# Autodesk Inventor assembly: Support
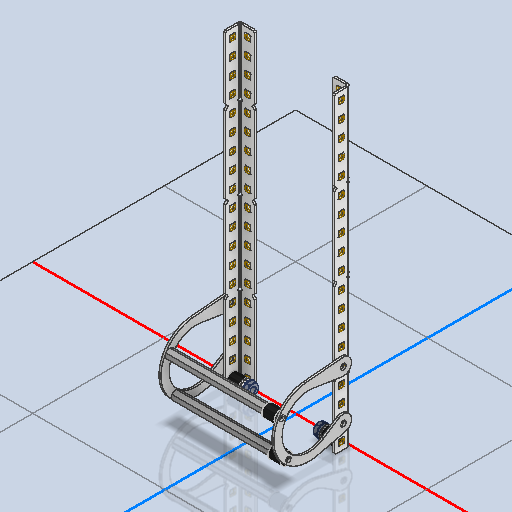
[picture p0: Inventor's stored thumbnail of the model, 512x512]
Saved by Autodesk Inventor 2026 (Build 300175000, 175)
## iProperties
Created: 2025-04-05
Part Number: Support
Document SubType Name: Assembly
Designer: avere
Author: avere
## Documents named in this file (10)
- C:\Users\avere\OneDrive\Documents\VEX-CAD\V5-CAD\Conveyer\Support.iam
- C:\Users\avere\OneDrive\Documents\VEX-CAD\VEX-CAD-Inventor\Structure\Angle\Aluminum 1x1\Alu Angle 1x1x19.ipt
- C:\Users\avere\OneDrive\Documents\VEX-CAD\VEX-CAD-Inventor\Motion\Spacers\Spacer Nylon .375 OD\NSpacer .375 OD x .375.ipt
- C:\Users\avere\OneDrive\Documents\VEX-CAD\VEX-CAD-Inventor\Motion\Spacers\Spacer Nylon .375 OD.ipt
- C:\Users\avere\OneDrive\Documents\VEX-CAD\VEX-CAD-Inventor\Motion\Spacers\Washer Teflon\TWasher .375 OD x .04000.ipt
- C:\Users\avere\OneDrive\Documents\VEX-CAD\VEX-CAD-Inventor\Motion\Spacers\Washer Teflon.ipt
- C:\Users\avere\OneDrive\Documents\VEX-CAD\VEX-CAD-Inventor\Structure\Hardware\Nut Keps.ipt
- C:\Users\avere\OneDrive\Documents\VEX-CAD\V5-CAD\Conveyer\Custom Parts\Reservoir Mount.ipt
- C:\Users\avere\OneDrive\Documents\VEX-CAD\VEX-CAD-Inventor\Structure\Standoff\Standoff 3.00.ipt
- C:\Users\avere\OneDrive\Documents\VEX-CAD\VEX-CAD-Inventor\Structure\Standoff.ipt
## Components (14 placed, 6 different names)
1. Alu Angle 1x1x19:1 — Mate:1, Mate:2, Flush:1, Insert:3, Insert:10, Mate:4
2. NSpacer .375 OD x .375:1 — Insert:3, Insert:4
3. TWasher .375 OD x .04000:1 — Insert:4, Insert:8
4. Alu Angle 1x1x19:2 — Flush:2, Mate:3, Flush:3, Insert:6
5. NSpacer .375 OD x .375:2 — Insert:6, Insert:7
6. TWasher .375 OD x .04000:2 — Insert:7, Insert:9
7. Nut Keps:1 — Insert:8
8. Nut Keps:2 — Insert:9
9. Reservoir Mount:1 — Insert:10, Mate:4
10. Reservoir Mount:2 — Insert:11, Insert:12
11. Standoff 3.00:1 — Insert:11, Insert:14
12. Standoff 3.00:2 — Insert:12, Insert:13
13. NSpacer .375 OD x .375:3 — Insert:13
14. NSpacer .375 OD x .375:4 — Insert:14
## Relationships (18: Insert 11, Mate 4, Flush 3)
- Mate:1 (41.275 mm): Alu Angle 1x1x19:1
- Mate:2: Alu Angle 1x1x19:1
- Flush:1 (-120.65 mm): Alu Angle 1x1x19:1
- Insert:3: Alu Angle 1x1x19:1 ↔ NSpacer .375 OD x .375:1
- Insert:4: NSpacer .375 OD x .375:1 ↔ TWasher .375 OD x .04000:1
- Flush:2 (-120.65 mm): Alu Angle 1x1x19:2
- Mate:3: Alu Angle 1x1x19:2
- Flush:3 (41.275 mm): Alu Angle 1x1x19:2
- Insert:6: Alu Angle 1x1x19:2 ↔ NSpacer .375 OD x .375:2
- Insert:7: NSpacer .375 OD x .375:2 ↔ TWasher .375 OD x .04000:2
- Insert:8 (1.5875 mm): TWasher .375 OD x .04000:1 ↔ Nut Keps:1
- Insert:9 (1.5875 mm): TWasher .375 OD x .04000:2 ↔ Nut Keps:2
- Insert:10: Alu Angle 1x1x19:1 ↔ Reservoir Mount:1
- Mate:4: Alu Angle 1x1x19:1 ↔ Reservoir Mount:1
- Insert:11: Reservoir Mount:2 ↔ Standoff 3.00:1
- Insert:12: Reservoir Mount:2 ↔ Standoff 3.00:2
- Insert:13: Standoff 3.00:2 ↔ NSpacer .375 OD x .375:3
- Insert:14: Standoff 3.00:1 ↔ NSpacer .375 OD x .375:4
